# Autodesk Inventor assembly: 000.002 - Крепеж мотора СБ
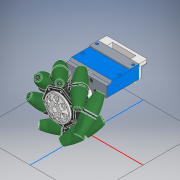
[picture p0: Inventor's stored thumbnail of the model, 180x180]
Saved by Autodesk Inventor 2022 (Build 260153000, 153)
## iProperties
Created: 2022-02-23
Part Number: 000.002 - Крепеж мотора СБ
Document SubType Name: Assembly
Designer: Petrov Ivan
Mass: 341.915 g
Surface Area: 2145.45 cm^2
Volume: 305.087 cm^3
Density: 1.12071 g/cm^3
Author: Petrov Ivan
## Documents named in this file (11)
- C:\Users\Ivan Petrov\Documents\GitHub\OmniBot\design\000.002 - Крепеж мотора СБ.iam
- C:\Users\Ivan Petrov\Documents\GitHub\OmniBot\design\000.002.001 - Крепеж мотора.ipt
- C:\Users\Ivan Petrov\Documents\GitHub\OmniBot\design\standart_components\vex_mechanum_adapter.ipt
- C:\Users\Ivan Petrov\Documents\GitHub\OmniBot\design\standart_components\Rueda 1.ipt
- C:\Users\Ivan Petrov\Documents\GitHub\OmniBot\design\standart_components\vex_mechanum_adapter (1) зеркальный.ipt
- C:\Users\Ivan Petrov\Documents\GitHub\OmniBot\design\Content Center Files\R2022\ru-RU\CSN 02 1143  B\CSN 02 1143 - M4 x 0,7 x 40(2).ipt
- C:\Users\Ivan Petrov\Documents\GitHub\OmniBot\design\standart_components\JGB37-520\JGB37-520.iam
- C:\Users\Ivan Petrov\Documents\GitHub\OmniBot\design\000.002.002 - Крышка мотора задняя.ipt
- C:\Users\Ivan Petrov\Documents\GitHub\OmniBot\design\Content Center Files\R2022\ru-RU\ANSI B18.6.3(29)\ANSI B18.6.3 - 6-32 UNC - 0,3125(13)135.ipt
- C:\Users\Ivan Petrov\Documents\GitHub\OmniBot\design\Content Center Files\R2022\ru-RU\IFI 513(1)\IFI 513 - M3x0,5 x 10(1) I.ipt
- C:\Users\Ivan Petrov\Documents\GitHub\OmniBot\design\000.002.003 - Металическая вставка.ipt
## Components (22 placed, 11 different names)
1. 000.002.001 - Крепеж мотора.ipt:1 — Совмещение:16, Угол:1, Совмещение:19, Совмещение:20, Угол:2, Заподлицо:4, Совмещение:21, Совмещение:22, Совмещение:23, Совмещение:24, Совмещение:25, Совмещение:26, Угол:3
2. vex_mechanum_adapter.ipt:1 — Совмещение:4, Совмещение:6, Совмещение:9, Совмещение:17, Совмещение:18, Совмещение:32, Заподлицо:5, Совмещение:36, Совмещение:37, Угол:4, Угол:5
3. Rueda 1.ipt:1 — Совмещение:4, Совмещение:6, Совмещение:7, Совмещение:8, Совмещение:34
4. vex_mechanum_adapter (1) зеркальный.ipt:1 — Совмещение:7, Совмещение:8, Совмещение:9, Совмещение:10, Совмещение:11, Совмещение:34
5. JGB37-520.iam:1 [sub-assembly] — Совмещение:16, Угол:1, Совмещение:17, Совмещение:18, Заподлицо:4, Угол:5
6. 000.002.002 - Крышка мотора задняя.ipt:1 — Совмещение:19, Совмещение:20, Угол:2, Вставка:1, Вставка:2
7. 000.002.003 - Металическая вставка:1 — Совмещение:36, Совмещение:37, Угол:4
8. ANSI B18.6.3 - 6-32 UNC - 0,3125(13)135.ipt:1 — Вставка:2
9. IFI 513 - M3x0,5 x 10(1) I.ipt:1 — Совмещение:21
10. IFI 513 - M3x0,5 x 10(1) I.ipt:2 — Совмещение:22
11. IFI 513 - M3x0,5 x 10(1) I.ipt:3 — Совмещение:23
12. IFI 513 - M3x0,5 x 10(1) I.ipt:4 — Совмещение:24
13. IFI 513 - M3x0,5 x 10(1) I.ipt:5 — Совмещение:25
14. IFI 513 - M3x0,5 x 10(1) I.ipt:6 — Совмещение:26
15. ANSI B18.6.3 - 6-32 UNC - 0,3125(13)135.ipt:2 — Вставка:1
16. CSN 02 1143 - M4 x 0,7 x 40(2).ipt:1 — Совмещение:10, Совмещение:11
17. CSN 02 1143 B M4 x 40:2
18. CSN 02 1143 B M4 x 40:3
19. CSN 02 1143 B M4 x 40:4
20. CSN 02 1143 B M4 x 40:5
21. CSN 02 1143 B M4 x 40:6
22. CSN 02 1143 B M4 x 40:7
## Component patterns: (7 elements, first: CSN 02 1143 - M4 x 0,7 x 40(2).ipt:1)
## Relationships (31: Mate 22, Angle 5, Insert 2, Flush 2)
- Совмещение:4 [Mate]: vex_mechanum_adapter.ipt:1 ↔ Rueda 1.ipt:1
- Совмещение:6 [Mate]: vex_mechanum_adapter.ipt:1 ↔ Rueda 1.ipt:1
- Совмещение:7 [Mate]: Rueda 1.ipt:1 ↔ vex_mechanum_adapter (1) зеркальный.ipt:1
- Совмещение:8 [Mate]: Rueda 1.ipt:1 ↔ vex_mechanum_adapter (1) зеркальный.ipt:1
- Совмещение:9 [Mate]: vex_mechanum_adapter.ipt:1 ↔ vex_mechanum_adapter (1) зеркальный.ipt:1
- Совмещение:10 [Mate]: vex_mechanum_adapter (1) зеркальный.ipt:1 ↔ CSN 02 1143 - M4 x 0,7 x 40(2).ipt:1
- Совмещение:11 [Mate]: vex_mechanum_adapter (1) зеркальный.ipt:1 ↔ CSN 02 1143 - M4 x 0,7 x 40(2).ipt:1
- Совмещение:16 [Mate]: 000.002.001 - Крепеж мотора.ipt:1 ↔ JGB37-520.iam:1
- Угол:1 [Angle] (90 deg): 000.002.001 - Крепеж мотора.ipt:1 ↔ JGB37-520.iam:1
- Совмещение:17 [Mate]: vex_mechanum_adapter.ipt:1 ↔ JGB37-520.iam:1
- Совмещение:18 [Mate]: vex_mechanum_adapter.ipt:1 ↔ JGB37-520.iam:1
- Совмещение:19 [Mate]: 000.002.001 - Крепеж мотора.ipt:1 ↔ 000.002.002 - Крышка мотора задняя.ipt:1
- Совмещение:20 [Mate]: 000.002.001 - Крепеж мотора.ipt:1 ↔ 000.002.002 - Крышка мотора задняя.ipt:1
- Угол:2 [Angle] (0 deg): 000.002.001 - Крепеж мотора.ipt:1 ↔ 000.002.002 - Крышка мотора задняя.ipt:1
- Вставка:1 [Insert]: 000.002.002 - Крышка мотора задняя.ipt:1 ↔ ANSI B18.6.3 - 6-32 UNC - 0,3125(13)135.ipt:2
- Вставка:2 [Insert]: 000.002.002 - Крышка мотора задняя.ipt:1 ↔ ANSI B18.6.3 - 6-32 UNC - 0,3125(13)135.ipt:1
- Заподлицо:4 [Flush]: 000.002.001 - Крепеж мотора.ipt:1 ↔ JGB37-520.iam:1
- Совмещение:21 [Mate]: 000.002.001 - Крепеж мотора.ipt:1 ↔ IFI 513 - M3x0,5 x 10(1) I.ipt:1
- Совмещение:22 [Mate]: 000.002.001 - Крепеж мотора.ipt:1 ↔ IFI 513 - M3x0,5 x 10(1) I.ipt:2
- Совмещение:23 [Mate]: 000.002.001 - Крепеж мотора.ipt:1 ↔ IFI 513 - M3x0,5 x 10(1) I.ipt:3
- Совмещение:24 [Mate]: 000.002.001 - Крепеж мотора.ipt:1 ↔ IFI 513 - M3x0,5 x 10(1) I.ipt:4
- Совмещение:25 [Mate]: 000.002.001 - Крепеж мотора.ipt:1 ↔ IFI 513 - M3x0,5 x 10(1) I.ipt:5
- Совмещение:26 [Mate]: 000.002.001 - Крепеж мотора.ipt:1 ↔ IFI 513 - M3x0,5 x 10(1) I.ipt:6
- Совмещение:32 [Mate]: vex_mechanum_adapter.ipt:1
- Заподлицо:5 [Flush]: vex_mechanum_adapter.ipt:1
- Совмещение:34 [Mate]: Rueda 1.ipt:1 ↔ vex_mechanum_adapter (1) зеркальный.ipt:1
- Угол:3 [Angle] (0 deg): 000.002.001 - Крепеж мотора.ipt:1
- Совмещение:36 [Mate]: vex_mechanum_adapter.ipt:1 ↔ 000.002.003 - Металическая вставка:1
- Совмещение:37 [Mate]: vex_mechanum_adapter.ipt:1 ↔ 000.002.003 - Металическая вставка:1
- Угол:4 [Angle] (180 deg): vex_mechanum_adapter.ipt:1 ↔ 000.002.003 - Металическая вставка:1
- Угол:5 [Angle] (0 deg): vex_mechanum_adapter.ipt:1 ↔ JGB37-520.iam:1
